# Autodesk Inventor assembly: pcb_assembly
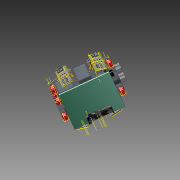
[picture p0: Inventor's stored thumbnail of the model, 180x180]
Saved by Autodesk Inventor 2014 (Build 180170000, 170)
## iProperties
Created: 2013-08-25
Part Number: pcb_assembly
Document SubType Name: Assembly
Designer: Felix
Author: Felix
## Documents named in this file (4)
- C:\Users\solidworks\Desktop\BEEP\Hardware\3D-CAD\parts\electronic\pcb_assembly.iam
- C:\Users\solidworks\Desktop\BEEP\Hardware\3D-CAD\parts\electronic\BEEP\beep_main_assembled.iam
- C:\Users\solidworks\Desktop\BEEP\Hardware\3D-CAD\parts\electronic\RaspberryPi\RaspberryPi.iam
- C:\Users\solidworks\Desktop\BEEP\Hardware\3D-CAD\parts\electronic\BEEP\beep_rgb_ir_assembled.iam
## Components (6 placed, 3 different names)
1. beep_main_assembled:1 [sub-assembly] — Passend:2, Passend:4, Passend:6, Passend:7, Passend:8, Passend:9, Passend:10, Passend:12, Passend:13, Fluchtend:1, Passend:16, Passend:17, Passend:18, Passend:19, Passend:20
2. RaspberryPi:1 [sub-assembly] — Passend:2, Passend:19, Passend:20
3. beep_rgb_ir_assembled:1 [sub-assembly] — Passend:4, Passend:6, Passend:7
4. beep_rgb_ir_assembled:2 [sub-assembly] — Passend:8, Passend:9, Passend:10
5. beep_rgb_ir_assembled:3 [sub-assembly] — Passend:16, Passend:17, Passend:18
6. beep_rgb_ir_assembled:4 [sub-assembly] — Passend:12, Passend:13, Fluchtend:1
## Relationships (15: Mate 14, Flush 1)
- Passend:2 [Mate]: beep_main_assembled:1 ↔ RaspberryPi:1
- Passend:4 [Mate]: beep_main_assembled:1 ↔ beep_rgb_ir_assembled:1
- Passend:6 [Mate]: beep_main_assembled:1 ↔ beep_rgb_ir_assembled:1
- Passend:7 [Mate]: beep_main_assembled:1 ↔ beep_rgb_ir_assembled:1
- Passend:8 [Mate]: beep_main_assembled:1 ↔ beep_rgb_ir_assembled:2
- Passend:9 [Mate]: beep_main_assembled:1 ↔ beep_rgb_ir_assembled:2
- Passend:10 [Mate]: beep_main_assembled:1 ↔ beep_rgb_ir_assembled:2
- Passend:12 [Mate]: beep_main_assembled:1 ↔ beep_rgb_ir_assembled:4
- Passend:13 [Mate]: beep_main_assembled:1 ↔ beep_rgb_ir_assembled:4
- Fluchtend:1 [Flush]: beep_main_assembled:1 ↔ beep_rgb_ir_assembled:4
- Passend:16 [Mate]: beep_main_assembled:1 ↔ beep_rgb_ir_assembled:3
- Passend:17 [Mate]: beep_main_assembled:1 ↔ beep_rgb_ir_assembled:3
- Passend:18 [Mate]: beep_main_assembled:1 ↔ beep_rgb_ir_assembled:3
- Passend:19 [Mate]: beep_main_assembled:1 ↔ RaspberryPi:1
- Passend:20 [Mate] (0.1 mm): beep_main_assembled:1 ↔ RaspberryPi:1
